# Autodesk Inventor assembly: Rod下
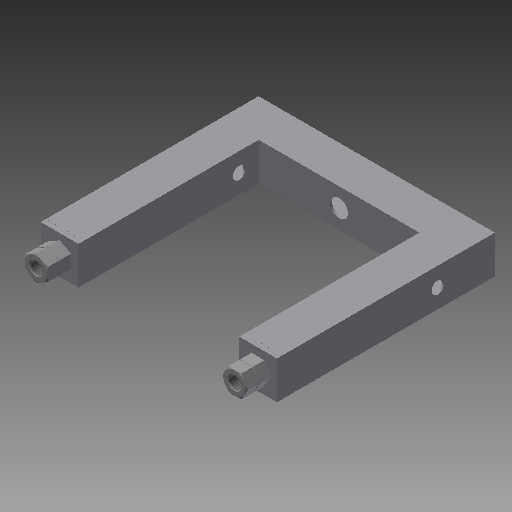
[picture p0: Inventor's stored thumbnail of the model, 512x512]
Saved by Autodesk Inventor 2018 (Build 220112000, 112)
## iProperties
Created: 2017-09-13
Part Number: Rod下
Material: 一般
Document SubType Name: Assembly
Designer: mura5
Author: mura5
## Documents named in this file (5)
- C:\Users\mura5\Documents\RBBR\cart\前足\Aアーム下.iam
- C:\Users\mura5\Documents\RBBR\cart\前足\PipeB穴あり.ipt
- C:\Users\mura5\Documents\RBBR\cart\前足\PipeB蓋.ipt
- C:\Users\mura5\Documents\RBBR\cart\前足\hn1_12.ipt
- C:\Users\mura5\Documents\RBBR\cart\前足\Pipe横.ipt
## Components (9 placed, 4 different names)
1. PipeB穴あり:1 — リジッド:4, リジッド:10
2. PipeB蓋:1 — リジッド:2, リジッド:10
3. hn1_12:1 — リジッド:2, リジッド:3
4. hn1_12:2 — リジッド:3
5. Pipe横:1 — リジッド:4, リジッド:5
6. PipeB穴あり:2 — リジッド:5, リジッド:9
7. PipeB蓋:2 — リジッド:7, リジッド:9
8. hn1_12:3 — リジッド:7, リジッド:8
9. hn1_12:4 — リジッド:8
## Relationships (8: WeldJoint 8)
- リジッド:2 [WeldJoint]: PipeB蓋:1 ↔ hn1_12:1
- リジッド:3 [WeldJoint]: hn1_12:1 ↔ hn1_12:2
- リジッド:4 [WeldJoint]: PipeB穴あり:1 ↔ Pipe横:1
- リジッド:5 [WeldJoint]: Pipe横:1 ↔ PipeB穴あり:2
- リジッド:7 [WeldJoint]: PipeB蓋:2 ↔ hn1_12:3
- リジッド:8 [WeldJoint]: hn1_12:3 ↔ hn1_12:4
- リジッド:9 [WeldJoint]: PipeB穴あり:2 ↔ PipeB蓋:2
- リジッド:10 [WeldJoint]: PipeB穴あり:1 ↔ PipeB蓋:1
